# Autodesk Inventor assembly: chest_piece_assembly
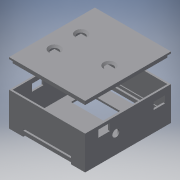
[picture p0: Inventor's stored thumbnail of the model, 180x180]
Saved by Autodesk Inventor 2017 (Build 210142000, 142)
## iProperties
Created: 2017-11-05
Part Number: chest_piece_assembly
Document SubType Name: Assembly
Designer: Gabe Madonna
Author: Gabe Madonna
## Documents named in this file (3)
- C:\Users\Gabe Madonna\Google Drive\MIT\Freshman\Spring\06.S08 Intro to EECS\6.S08_final\main\CAD Model\chest_piece_assembly.iam
- C:\Users\Gabe Madonna\Google Drive\MIT\Freshman\Spring\06.S08 Intro to EECS\6.S08_final\main\CAD Model\chest_piece_bottom_2.ipt
- C:\Users\Gabe Madonna\Google Drive\MIT\Freshman\Spring\06.S08 Intro to EECS\6.S08_final\main\CAD Model\chest_piece_top_2.ipt
## Components (2 placed, 2 different names)
1. chest_piece_bottom_2:1 — Mate:1, Mate:2, Mate:3
2. chest_piece_top_2:1 — Mate:1, Mate:2, Mate:3
## Relationships (3: Mate 3)
- Mate:1: chest_piece_bottom_2:1 ↔ chest_piece_top_2:1
- Mate:2: chest_piece_bottom_2:1 ↔ chest_piece_top_2:1
- Mate:3: chest_piece_bottom_2:1 ↔ chest_piece_top_2:1
